# Autodesk Inventor assembly: Main_assssembly
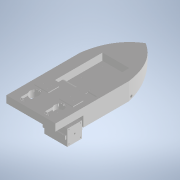
[picture p0: Inventor's stored thumbnail of the model, 180x180]
Saved by Autodesk Inventor 2020.1 (Build 241239000, 239)
## iProperties
Created: 2022-02-07
Part Number: Main_assssembly
Document SubType Name: Assembly
Designer: OEM
Author: OEM
## Documents named in this file (6)
- D:\Studia\Bobr\Repo\CAD\Main_assssembly.iam
- D:\Studia\Bobr\Repo\CAD\MainBody.ipt
- D:\Studia\Bobr\Repo\CAD\connector_sleeve.ipt
- D:\Studia\Bobr\Repo\CAD\engine_sleeve_full.ipt
- D:\Studia\Bobr\Repo\CAD\engine_cup.ipt
- D:\Studia\Bobr\Repo\CAD\engine_lid.ipt
## Components (5 placed, 5 different names)
1. MainBody:2 — Rotational:1
2. connector_sleeve:1 — Rotational:1, Mate:1
3. engine_sleeve_full:1 — Mate:1, Mate:2, Mate:3, Mate:4
4. engine_cup:1 — Mate:2, Mate:3
5. engine_lid:1 — Mate:4
## Relationships (5: Mate 4, RevoluteJoint 1)
- Rotational:1 [RevoluteJoint]: MainBody:2 ↔ connector_sleeve:1
- Mate:1: connector_sleeve:1 ↔ engine_sleeve_full:1
- Mate:2: engine_sleeve_full:1 ↔ engine_cup:1
- Mate:3: engine_sleeve_full:1 ↔ engine_cup:1
- Mate:4: engine_sleeve_full:1 ↔ engine_lid:1
